# Autodesk Inventor assembly: Shooter Assembly
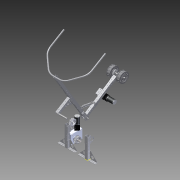
[picture p0: Inventor's stored thumbnail of the model, 180x180]
Saved by Autodesk Inventor 2014 (Build 180170000, 170)
## iProperties
Created: 2014-01-05
Part Number: Shooter Assembly
Document SubType Name: Assembly
Designer: Andrew Toennies
Mass: 7781.82 g
Surface Area: 22307.5 cm^2
Volume: 3128.72 cm^3
Density: 2.48722 g/cm^3
Author: Andrew Toennies
## Documents named in this file (34)
- C:\Users\Andrew Toennies\Documents\GitHub\2014buildCAD\Shooter\Shooter Assembly.iam
- C:\Users\Andrew Toennies\Documents\GitHub\2014buildCAD\Shooter\Vex Pro 1x1 rectangular tubing 12 in length.ipt
- C:\Users\Andrew Toennies\Documents\GitHub\2014buildCAD\Shooter\Vex Pro End Bearing Mount.ipt
- C:\Users\Andrew Toennies\Documents\GitHub\2014buildCAD\Shooter\Vex Pro 1x1 rectangular tubing 27 in length.ipt
- C:\Users\Andrew Toennies\Documents\GitHub\2014buildCAD\Shooter\Vex Pro 1x1 rectangular tubing 24 in length.ipt
- C:\Users\Andrew Toennies\Documents\GitHub\2014buildCAD\Shooter\Vex Pro Corner Gusset.ipt
- C:\Users\Andrew Toennies\Documents\GitHub\2014buildCAD\Shooter\Vex Pro 1x1 rectangular tubing 13 in length.ipt
- C:\Users\Andrew Toennies\Documents\GitHub\2014buildCAD\Shooter\Bearing ID 0.500 Hex OD 1.125.ipt
- C:\Users\Andrew Toennies\Documents\GitHub\2014buildCAD\Shooter\Axle 0.500 Hex 5 in length.ipt
- C:\Users\Andrew Toennies\Documents\GitHub\2014buildCAD\Shooter\Spacer.ipt
- C:\Users\Andrew Toennies\Documents\GitHub\2014buildCAD\Shooter\Bearing ID 0.375 OD 1.125.ipt
- C:\Users\Andrew Toennies\Documents\GitHub\2014buildCAD\Shooter\Axle 0.375 3 in length.ipt
- C:\Users\Andrew Toennies\Documents\GitHub\2014buildCAD\Shooter\Vex Pro 30 tooth 9mm timing belt pulley.ipt
- C:\Users\Andrew Toennies\Documents\GitHub\2014buildCAD\Shooter\Vex Pro VersaHub 0.500 Hex.ipt
- C:\Users\Andrew Toennies\Documents\GitHub\2014buildCAD\Shooter\Axle 0.500 Hex 3 in length.ipt
- C:\Users\Andrew Toennies\Documents\GitHub\2014buildCAD\Shooter\Worm-Drive-Gearbox-16to1.iam
- C:\Users\Andrew Toennies\Documents\GitHub\2014buildCAD\Shooter\Vex Pro 32 tooth 15 mm timing belt pulley.ipt
- C:\Users\Andrew Toennies\Documents\GitHub\2014buildCAD\Shooter\Vex Pro Traction 1 in wide 4 in dia wheel.iam
- C:\Users\Andrew Toennies\Documents\GitHub\2014buildCAD\Shooter\Aluminum Tube Bent 0.500 OD 0.436 ID.ipt
- C:\Users\Andrew Toennies\Documents\GitHub\2014buildCAD\Shooter\Bag Motor with VersaPlanetary 10 to 1 Reduction.iam
- C:\Users\Andrew Toennies\Documents\GitHub\2014buildCAD\Shooter\Vex Pro 18 tooth timing belt pulley.ipt
- C:\Users\Andrew Toennies\Documents\GitHub\2014buildCAD\Shooter\Vex Pro VersaPlanetary Face Mount.ipt
- C:\Users\Andrew Toennies\Documents\GitHub\2014buildCAD\Shooter\Foot Bracket Mount (McMaster Part #6498K710).ipt
- C:\Users\Andrew Toennies\Documents\GitHub\2014buildCAD\Shooter\Rod End (McMaster Part #6498K592).ipt
- C:\Users\Andrew Toennies\Documents\GitHub\2014buildCAD\Shooter\Spacer2.ipt
- C:\Users\Andrew Toennies\Documents\GitHub\2014buildCAD\Shooter\Bracket.ipt
- C:\Users\Andrew Toennies\Documents\GitHub\2014buildCAD\Shooter\Vex Pro 1x1 rectangular tubing 2 in length.ipt
- C:\Users\Andrew Toennies\Documents\GitHub\2014buildCAD\Shooter\Waterjetted Face Mount Bearing support VersaPlanetary.ipt
- C:\Users\Andrew Toennies\Documents\GitHub\2014buildCAD\Shooter\Axle 0.190 in 3 in length.ipt
- C:\Users\Andrew Toennies\Documents\GitHub\2014buildCAD\Shooter\6498K602 Pneumatic Cylinder Assembly.iam
- C:\Users\Andrew Toennies\Documents\GitHub\2014buildCAD\Shooter\mcmaster carr 32 tooth pulley.ipt
- C:\Users\Andrew Toennies\Documents\GitHub\2014buildCAD\Shooter\Vex Pro 1x1 rectangular tubing 4 in length.ipt
- C:\Users\Andrew Toennies\Documents\GitHub\2014buildCAD\Shooter\Vex Pro VersaFrame 90 Degree.ipt
- C:\Users\Andrew Toennies\Documents\GitHub\2014buildCAD\Shooter\Ball.ipt
## Components (59 placed, 33 different names)
1. Vex Pro Corner Gusset:1 — Insert:9, Insert:10, Mate:217, Flush:60, Flush:61
2. Vex Pro Corner Gusset:2 — Insert:11, Insert:12, Flush:50, Mate:216, Flush:78
3. Vex Pro End Bearing Mount:3 — Insert:35, Insert:47, Insert:48
4. Vex Pro End Bearing Mount:4 — Insert:36, Insert:49, Insert:50
5. Vex Pro End Bearing Mount:5 — Insert:21, Insert:22, Insert:25
6. Vex Pro End Bearing Mount:6 — Insert:23, Insert:24, Insert:26
7. Bearing ID 0.500 Hex OD 1.125:1 — Insert:26, Flush:7, Mate:7, Mate:8
8. Bearing ID 0.500 Hex OD 1.125:2 — Insert:25, Flush:7, Mate:16
9. Axle 0.500 Hex 5 in length:1 — Mate:7, Mate:8, Flush:8, Mate:14, Mate:15, Mate:18, Mate:19, Mate:21, Mate:22, Flush:12, Flush:16
10. Spacer:1 — Insert:47, Insert:48, Mate:65, Flush:24
11. Spacer:2 — Insert:49, Insert:50, Flush:22, Flush:23, Mate:64
12. Bearing ID 0.375 OD 1.125:1 — Insert:35, Mate:9
13. Bearing ID 0.375 OD 1.125:2 — Insert:36, Mate:66
14. Axle 0.375 3 in length:1 — Mate:9, Flush:9, Mate:66, Mate:85
15. Vex Pro 30 tooth 9mm timing belt pulley:1 — Mate:14, Mate:15, Mate:16, Flush:18
16. Vex Pro VersaHub 0.500 Hex:1 — Mate:17, Mate:18, Mate:19, Flush:16, Insert:51, Mate:105
17. Vex Pro VersaHub 0.500 Hex:2 — Mate:17, Mate:105
18. Vex Pro VersaHub 0.500 Hex:3 — Mate:20, Mate:21, Mate:22, Flush:12, Mate:52, Insert:64
19. Vex Pro VersaHub 0.500 Hex:4 — Mate:20, Mate:52, Insert:52
20. Axle 0.500 Hex 3 in length:1 — Mate:47, Mate:48, Mate:210, Mate:211, Flush:58, Flush:59
21. Worm-Drive-Gearbox-16to1:1 [sub-assembly] — Mate:49, Mate:50, Mate:170, Mate:196
22. Vex Pro 32 tooth 15 mm timing belt pulley:1 — Mate:47, Mate:48, Flush:40, Rotation:1
23. Vex Pro Traction 1 in wide 4 in dia wheel:1 [sub-assembly] — Insert:51
24. Vex Pro Traction 1 in wide 4 in dia wheel:2 [sub-assembly] — Insert:52, Insert:64
25. Aluminum Tube Bent 0.500 OD 0.436 ID:1 — Mate:53, Tangent:1, Tangent:2, Mate:230, Flush:80
26. Bag Motor with VersaPlanetary 10 to 1 Reduction:1 [sub-assembly] — Mate:55, Mate:56, Flush:19, Insert:53, Insert:54, Angle:4
27. Vex Pro 18 tooth timing belt pulley:1 — Mate:55, Mate:56, Flush:18
28. Vex Pro VersaPlanetary Face Mount:1 — Insert:53, Insert:54, Flush:21, Mate:63, Mate:77, Mate:78, Mate:79
29. Foot Bracket Mount (McMaster Part #6498K710):1 — Mate:71, Mate:72, Mate:73, Mate:99, Mate:100
30. Rod End (McMaster Part #6498K592):1 — Mate:102, Mate:103, Mate:194
31. Spacer2:1 — Mate:71, Mate:72, Mate:73, Mate:84, Mate:229
32. Bracket:1 — Mate:93, Mate:96, Flush:25, Flush:28, Flush:29
33. Bracket:2 — Mate:86, Mate:97, Flush:26, Flush:27
34. Waterjetted Face Mount Bearing support VersaPlanetary:1 — Mate:80, Mate:81, Mate:82, Insert:63
35. Bearing ID 0.500 Hex OD 1.125:5 — Insert:63, Angle:4
36. Axle 0.190 in 3 in length:1 — Mate:96, Mate:97, Flush:25, Mate:103
37. 6498K602 Pneumatic Cylinder Assembly:1 [sub-assembly] — Mate:99, Mate:100, Mate:102, Mate:194
38. mcmaster carr 32 tooth pulley:1 — Mate:170, Flush:40, Rotation:1
39. Vex Pro Corner Gusset:6 — Mate:182, Mate:183, Flush:45, Mate:231
40. Vex Pro Corner Gusset:7 — Flush:49, Flush:50, Mate:216, Mate:220, Flush:68, Flush:78
41. Vex Pro Corner Gusset:8 — Flush:49, Mate:221, Flush:68, Flush:69, Flush:70
42. Bearing ID 0.500 Hex OD 1.125:4 — Flush:57, Mate:210, Flush:59
43. Bearing ID 0.500 Hex OD 1.125:3 — Flush:55
44. Bearing ID 0.500 Hex OD 1.125:6 — Flush:55, Flush:56, Flush:58
45. Bearing ID 0.500 Hex OD 1.125:7 — Flush:56, Flush:57, Mate:211
46. Vex Pro Corner Gusset:9 — Mate:217, Flush:60, Flush:61, Flush:64, Flush:65, Mate:218, Flush:66, Flush:67
47. Vex Pro Corner Gusset:10 — Flush:64, Flush:65, Mate:219
48. Vex Pro VersaFrame 90 Degree:1 — Mate:222, Flush:71, Mate:223, Mate:227
49. Vex Pro VersaFrame 90 Degree:2 — Mate:224, Flush:72, Flush:73
50. Vex Pro VersaFrame 90 Degree:3 — Mate:225, Flush:74, Flush:75
51. Vex Pro VersaFrame 90 Degree:4 — Mate:226, Flush:76, Flush:77
52. Ball:1 — Tangent:1, Tangent:2
53. Vex Pro 1x1 rectangular tubing 2 in length:1 — Mate:77, Mate:78, Mate:79, Mate:80, Mate:81, Mate:82
54. Vex Pro 1x1 rectangular tubing 4 in length:2 — Mate:220, Mate:221, Flush:69, Flush:70, Mate:222, Flush:71, Mate:223, Mate:224, Flush:72, Flush:73
55. Vex Pro 1x1 rectangular tubing 4 in length:1 — Mate:218, Flush:66, Flush:67, Mate:219, Mate:225, Flush:74, Flush:75, Mate:226, Flush:76, Flush:77
56. Vex Pro 1x1 rectangular tubing 12 in length:1 — Insert:9, Insert:10, Insert:11, Insert:12, Mate:49, Mate:50, Mate:196
57. Vex Pro 1x1 rectangular tubing 27 in length:1 — Flush:2, Mate:2, Mate:182, Flush:45, Mate:227
58. Vex Pro 1x1 rectangular tubing 24 in length:1 — Flush:2, Mate:2, Flush:3, Flush:9, Mate:53, Flush:22, Flush:23, Mate:64, Mate:65, Flush:24, Mate:84, Mate:183, Mate:229, Mate:230, Mate:231, Flush:79
59. Vex Pro 1x1 rectangular tubing 13 in length:1 — Flush:3, Insert:21, Insert:22, Insert:23, Insert:24, Flush:8, Flush:19, Flush:21, Mate:63, Mate:85, Mate:86, Mate:93, Flush:26, Flush:27, Flush:28, Flush:29
## Relationships (139: Mate 67, Flush 46, Insert 22, Tangent 2, Angle 1, RelateRotation 1)
- Flush:2: Vex Pro 1x1 rectangular tubing 27 in length:1 ↔ Vex Pro 1x1 rectangular tubing 24 in length:1
- Mate:2: Vex Pro 1x1 rectangular tubing 27 in length:1 ↔ Vex Pro 1x1 rectangular tubing 24 in length:1
- Insert:9: Vex Pro Corner Gusset:1 ↔ Vex Pro 1x1 rectangular tubing 12 in length:1
- Insert:10: Vex Pro Corner Gusset:1 ↔ Vex Pro 1x1 rectangular tubing 12 in length:1
- Insert:11: Vex Pro Corner Gusset:2 ↔ Vex Pro 1x1 rectangular tubing 12 in length:1
- Insert:12: Vex Pro Corner Gusset:2 ↔ Vex Pro 1x1 rectangular tubing 12 in length:1
- Flush:3: Vex Pro 1x1 rectangular tubing 24 in length:1 ↔ Vex Pro 1x1 rectangular tubing 13 in length:1
- Insert:21: Vex Pro End Bearing Mount:5 ↔ Vex Pro 1x1 rectangular tubing 13 in length:1
- Insert:22: Vex Pro End Bearing Mount:5 ↔ Vex Pro 1x1 rectangular tubing 13 in length:1
- Insert:23: Vex Pro End Bearing Mount:6 ↔ Vex Pro 1x1 rectangular tubing 13 in length:1
- Insert:24: Vex Pro End Bearing Mount:6 ↔ Vex Pro 1x1 rectangular tubing 13 in length:1
- Insert:25: Vex Pro End Bearing Mount:5 ↔ Bearing ID 0.500 Hex OD 1.125:2
- Insert:26: Vex Pro End Bearing Mount:6 ↔ Bearing ID 0.500 Hex OD 1.125:1
- Flush:7: Bearing ID 0.500 Hex OD 1.125:1 ↔ Bearing ID 0.500 Hex OD 1.125:2
- Mate:7: Bearing ID 0.500 Hex OD 1.125:1 ↔ Axle 0.500 Hex 5 in length:1
- Mate:8: Bearing ID 0.500 Hex OD 1.125:1 ↔ Axle 0.500 Hex 5 in length:1
- Flush:8 (-63.5 mm): Axle 0.500 Hex 5 in length:1 ↔ Vex Pro 1x1 rectangular tubing 13 in length:1
- Insert:35: Vex Pro End Bearing Mount:3 ↔ Bearing ID 0.375 OD 1.125:1
- Insert:36: Vex Pro End Bearing Mount:4 ↔ Bearing ID 0.375 OD 1.125:2
- Mate:9: Bearing ID 0.375 OD 1.125:1 ↔ Axle 0.375 3 in length:1
- Flush:9 (-25.4 mm): Axle 0.375 3 in length:1 ↔ Vex Pro 1x1 rectangular tubing 24 in length:1
- Mate:14: Axle 0.500 Hex 5 in length:1 ↔ Vex Pro 30 tooth 9mm timing belt pulley:1
- Mate:15: Axle 0.500 Hex 5 in length:1 ↔ Vex Pro 30 tooth 9mm timing belt pulley:1
- Mate:16: Bearing ID 0.500 Hex OD 1.125:2 ↔ Vex Pro 30 tooth 9mm timing belt pulley:1
- Mate:17: Vex Pro VersaHub 0.500 Hex:1 ↔ Vex Pro VersaHub 0.500 Hex:2
- Mate:18: Axle 0.500 Hex 5 in length:1 ↔ Vex Pro VersaHub 0.500 Hex:1
- Mate:19: Axle 0.500 Hex 5 in length:1 ↔ Vex Pro VersaHub 0.500 Hex:1
- Mate:20: Vex Pro VersaHub 0.500 Hex:3 ↔ Vex Pro VersaHub 0.500 Hex:4
- Mate:21: Axle 0.500 Hex 5 in length:1 ↔ Vex Pro VersaHub 0.500 Hex:3
- Mate:22: Axle 0.500 Hex 5 in length:1 ↔ Vex Pro VersaHub 0.500 Hex:3
- Flush:12 (9.525 mm): Axle 0.500 Hex 5 in length:1 ↔ Vex Pro VersaHub 0.500 Hex:3
- Flush:16 (12.7 mm): Axle 0.500 Hex 5 in length:1 ↔ Vex Pro VersaHub 0.500 Hex:1
- Mate:47: Axle 0.500 Hex 3 in length:1 ↔ Vex Pro 32 tooth 15 mm timing belt pulley:1
- Mate:48: Axle 0.500 Hex 3 in length:1 ↔ Vex Pro 32 tooth 15 mm timing belt pulley:1
- Mate:49: Worm-Drive-Gearbox-16to1:1 ↔ Vex Pro 1x1 rectangular tubing 12 in length:1
- Mate:50: Worm-Drive-Gearbox-16to1:1 ↔ Vex Pro 1x1 rectangular tubing 12 in length:1
- Insert:47: Vex Pro End Bearing Mount:3 ↔ Spacer:1
- Insert:48: Vex Pro End Bearing Mount:3 ↔ Spacer:1
- Insert:49: Vex Pro End Bearing Mount:4 ↔ Spacer:2
- Insert:50: Vex Pro End Bearing Mount:4 ↔ Spacer:2
- Mate:52: Vex Pro VersaHub 0.500 Hex:3 ↔ Vex Pro VersaHub 0.500 Hex:4
- Insert:51: Vex Pro VersaHub 0.500 Hex:1 ↔ Vex Pro Traction 1 in wide 4 in dia wheel:1
- Insert:52: Vex Pro VersaHub 0.500 Hex:4 ↔ Vex Pro Traction 1 in wide 4 in dia wheel:2
- Mate:53: Aluminum Tube Bent 0.500 OD 0.436 ID:1 ↔ Vex Pro 1x1 rectangular tubing 24 in length:1
- Mate:55: Bag Motor with VersaPlanetary 10 to 1 Reduction:1 ↔ Vex Pro 18 tooth timing belt pulley:1
- Mate:56: Bag Motor with VersaPlanetary 10 to 1 Reduction:1 ↔ Vex Pro 18 tooth timing belt pulley:1
- Flush:18: Vex Pro 30 tooth 9mm timing belt pulley:1 ↔ Vex Pro 18 tooth timing belt pulley:1
- Flush:19: Bag Motor with VersaPlanetary 10 to 1 Reduction:1 ↔ Vex Pro 1x1 rectangular tubing 13 in length:1
- Insert:53: Bag Motor with VersaPlanetary 10 to 1 Reduction:1 ↔ Vex Pro VersaPlanetary Face Mount:1
- Insert:54: Bag Motor with VersaPlanetary 10 to 1 Reduction:1 ↔ Vex Pro VersaPlanetary Face Mount:1
- Flush:21: Vex Pro VersaPlanetary Face Mount:1 ↔ Vex Pro 1x1 rectangular tubing 13 in length:1
- Mate:63: Vex Pro VersaPlanetary Face Mount:1 ↔ Vex Pro 1x1 rectangular tubing 13 in length:1
- Flush:22: Spacer:2 ↔ Vex Pro 1x1 rectangular tubing 24 in length:1
- Flush:23: Spacer:2 ↔ Vex Pro 1x1 rectangular tubing 24 in length:1
- Mate:64: Spacer:2 ↔ Vex Pro 1x1 rectangular tubing 24 in length:1
- Mate:65: Spacer:1 ↔ Vex Pro 1x1 rectangular tubing 24 in length:1
- Flush:24: Spacer:1 ↔ Vex Pro 1x1 rectangular tubing 24 in length:1
- Mate:66: Bearing ID 0.375 OD 1.125:2 ↔ Axle 0.375 3 in length:1
- Mate:71: Foot Bracket Mount (McMaster Part #6498K710):1 ↔ Spacer2:1
- Mate:72: Foot Bracket Mount (McMaster Part #6498K710):1 ↔ Spacer2:1
- Mate:73: Foot Bracket Mount (McMaster Part #6498K710):1 ↔ Spacer2:1
- Mate:77: Vex Pro VersaPlanetary Face Mount:1 ↔ Vex Pro 1x1 rectangular tubing 2 in length:1
- Mate:78: Vex Pro VersaPlanetary Face Mount:1 ↔ Vex Pro 1x1 rectangular tubing 2 in length:1
- Mate:79: Vex Pro VersaPlanetary Face Mount:1 ↔ Vex Pro 1x1 rectangular tubing 2 in length:1
- Mate:80: Waterjetted Face Mount Bearing support VersaPlanetary:1 ↔ Vex Pro 1x1 rectangular tubing 2 in length:1
- Mate:81: Waterjetted Face Mount Bearing support VersaPlanetary:1 ↔ Vex Pro 1x1 rectangular tubing 2 in length:1
- Mate:82: Waterjetted Face Mount Bearing support VersaPlanetary:1 ↔ Vex Pro 1x1 rectangular tubing 2 in length:1
- Insert:63: Waterjetted Face Mount Bearing support VersaPlanetary:1 ↔ Bearing ID 0.500 Hex OD 1.125:5
- Angle:4 (0 deg): Bag Motor with VersaPlanetary 10 to 1 Reduction:1 ↔ Bearing ID 0.500 Hex OD 1.125:5
- Mate:84: Spacer2:1 ↔ Vex Pro 1x1 rectangular tubing 24 in length:1
- Insert:64: Vex Pro VersaHub 0.500 Hex:3 ↔ Vex Pro Traction 1 in wide 4 in dia wheel:2
- Mate:85: Axle 0.375 3 in length:1 ↔ Vex Pro 1x1 rectangular tubing 13 in length:1
- Mate:86: Bracket:2 ↔ Vex Pro 1x1 rectangular tubing 13 in length:1
- Mate:93: Bracket:1 ↔ Vex Pro 1x1 rectangular tubing 13 in length:1
- Mate:96: Bracket:1 ↔ Axle 0.190 in 3 in length:1
- Mate:97: Bracket:2 ↔ Axle 0.190 in 3 in length:1
- Flush:25 (-11.1125 mm): Bracket:1 ↔ Axle 0.190 in 3 in length:1
- Flush:26: Bracket:2 ↔ Vex Pro 1x1 rectangular tubing 13 in length:1
- Flush:27 (109.22 mm): Bracket:2 ↔ Vex Pro 1x1 rectangular tubing 13 in length:1
- Flush:28 (109.22 mm): Bracket:1 ↔ Vex Pro 1x1 rectangular tubing 13 in length:1
- Flush:29: Bracket:1 ↔ Vex Pro 1x1 rectangular tubing 13 in length:1
- Mate:99: Foot Bracket Mount (McMaster Part #6498K710):1 ↔ 6498K602 Pneumatic Cylinder Assembly:1
- Mate:100: Foot Bracket Mount (McMaster Part #6498K710):1 ↔ 6498K602 Pneumatic Cylinder Assembly:1
- Mate:102: Rod End (McMaster Part #6498K592):1 ↔ 6498K602 Pneumatic Cylinder Assembly:1
- Mate:103: Rod End (McMaster Part #6498K592):1 ↔ Axle 0.190 in 3 in length:1
- Mate:105: Vex Pro VersaHub 0.500 Hex:1 ↔ Vex Pro VersaHub 0.500 Hex:2
- Mate:170: Worm-Drive-Gearbox-16to1:1 ↔ mcmaster carr 32 tooth pulley:1
- Flush:40: Vex Pro 32 tooth 15 mm timing belt pulley:1 ↔ mcmaster carr 32 tooth pulley:1
- Rotation:1 [RelateRotation] (1 ul): Vex Pro 32 tooth 15 mm timing belt pulley:1 ↔ mcmaster carr 32 tooth pulley:1
- Mate:182: Vex Pro Corner Gusset:6 ↔ Vex Pro 1x1 rectangular tubing 27 in length:1
- Mate:183: Vex Pro Corner Gusset:6 ↔ Vex Pro 1x1 rectangular tubing 24 in length:1
- Flush:45: Vex Pro Corner Gusset:6 ↔ Vex Pro 1x1 rectangular tubing 27 in length:1
- Mate:194 (-12.7 mm): Rod End (McMaster Part #6498K592):1 ↔ 6498K602 Pneumatic Cylinder Assembly:1
- Mate:196: Worm-Drive-Gearbox-16to1:1 ↔ Vex Pro 1x1 rectangular tubing 12 in length:1
- Flush:49: Vex Pro Corner Gusset:7 ↔ Vex Pro Corner Gusset:8
- Flush:50: Vex Pro Corner Gusset:2 ↔ Vex Pro Corner Gusset:7
- Flush:55: Bearing ID 0.500 Hex OD 1.125:3 ↔ Bearing ID 0.500 Hex OD 1.125:6
- Flush:56: Bearing ID 0.500 Hex OD 1.125:6 ↔ Bearing ID 0.500 Hex OD 1.125:7
- Flush:57: Bearing ID 0.500 Hex OD 1.125:4 ↔ Bearing ID 0.500 Hex OD 1.125:7
- Mate:210: Axle 0.500 Hex 3 in length:1 ↔ Bearing ID 0.500 Hex OD 1.125:4
- Mate:211: Axle 0.500 Hex 3 in length:1 ↔ Bearing ID 0.500 Hex OD 1.125:7
- Flush:58: Axle 0.500 Hex 3 in length:1 ↔ Bearing ID 0.500 Hex OD 1.125:6
- Flush:59: Axle 0.500 Hex 3 in length:1 ↔ Bearing ID 0.500 Hex OD 1.125:4
- Mate:216 (50.8 mm): Vex Pro Corner Gusset:2 ↔ Vex Pro Corner Gusset:7
- Mate:217: Vex Pro Corner Gusset:1 ↔ Vex Pro Corner Gusset:9
- Flush:60: Vex Pro Corner Gusset:1 ↔ Vex Pro Corner Gusset:9
- Flush:61: Vex Pro Corner Gusset:1 ↔ Vex Pro Corner Gusset:9
- Flush:64: Vex Pro Corner Gusset:9 ↔ Vex Pro Corner Gusset:10
- Flush:65: Vex Pro Corner Gusset:9 ↔ Vex Pro Corner Gusset:10
- Mate:218: Vex Pro Corner Gusset:9 ↔ Vex Pro 1x1 rectangular tubing 4 in length:1
- Flush:66: Vex Pro Corner Gusset:9 ↔ Vex Pro 1x1 rectangular tubing 4 in length:1
- Flush:67: Vex Pro Corner Gusset:9 ↔ Vex Pro 1x1 rectangular tubing 4 in length:1
- Mate:219: Vex Pro Corner Gusset:10 ↔ Vex Pro 1x1 rectangular tubing 4 in length:1
- Mate:220: Vex Pro Corner Gusset:7 ↔ Vex Pro 1x1 rectangular tubing 4 in length:2
- Mate:221: Vex Pro Corner Gusset:8 ↔ Vex Pro 1x1 rectangular tubing 4 in length:2
- Flush:68: Vex Pro Corner Gusset:7 ↔ Vex Pro Corner Gusset:8
- Flush:69: Vex Pro Corner Gusset:8 ↔ Vex Pro 1x1 rectangular tubing 4 in length:2
- Flush:70: Vex Pro Corner Gusset:8 ↔ Vex Pro 1x1 rectangular tubing 4 in length:2
- Mate:222: Vex Pro VersaFrame 90 Degree:1 ↔ Vex Pro 1x1 rectangular tubing 4 in length:2
- Flush:71: Vex Pro VersaFrame 90 Degree:1 ↔ Vex Pro 1x1 rectangular tubing 4 in length:2
- Mate:223: Vex Pro VersaFrame 90 Degree:1 ↔ Vex Pro 1x1 rectangular tubing 4 in length:2
- Mate:224: Vex Pro VersaFrame 90 Degree:2 ↔ Vex Pro 1x1 rectangular tubing 4 in length:2
- Flush:72: Vex Pro VersaFrame 90 Degree:2 ↔ Vex Pro 1x1 rectangular tubing 4 in length:2
- Flush:73: Vex Pro VersaFrame 90 Degree:2 ↔ Vex Pro 1x1 rectangular tubing 4 in length:2
- Mate:225: Vex Pro VersaFrame 90 Degree:3 ↔ Vex Pro 1x1 rectangular tubing 4 in length:1
- Flush:74: Vex Pro VersaFrame 90 Degree:3 ↔ Vex Pro 1x1 rectangular tubing 4 in length:1
- Flush:75: Vex Pro VersaFrame 90 Degree:3 ↔ Vex Pro 1x1 rectangular tubing 4 in length:1
- Mate:226: Vex Pro VersaFrame 90 Degree:4 ↔ Vex Pro 1x1 rectangular tubing 4 in length:1
- Flush:76: Vex Pro VersaFrame 90 Degree:4 ↔ Vex Pro 1x1 rectangular tubing 4 in length:1
- Flush:77: Vex Pro VersaFrame 90 Degree:4 ↔ Vex Pro 1x1 rectangular tubing 4 in length:1
- Mate:227: Vex Pro VersaFrame 90 Degree:1 ↔ Vex Pro 1x1 rectangular tubing 27 in length:1
- Flush:78: Vex Pro Corner Gusset:2 ↔ Vex Pro Corner Gusset:7
- Tangent:1: Aluminum Tube Bent 0.500 OD 0.436 ID:1 ↔ Ball:1
- Tangent:2: Aluminum Tube Bent 0.500 OD 0.436 ID:1 ↔ Ball:1
- Mate:229: Spacer2:1 ↔ Vex Pro 1x1 rectangular tubing 24 in length:1
- Mate:230 (-12.7 mm): Aluminum Tube Bent 0.500 OD 0.436 ID:1 ↔ Vex Pro 1x1 rectangular tubing 24 in length:1
- Mate:231: Vex Pro Corner Gusset:6 ↔ Vex Pro 1x1 rectangular tubing 24 in length:1
- Flush:79 (330.2 mm): Vex Pro 1x1 rectangular tubing 24 in length:1
- Flush:80: Aluminum Tube Bent 0.500 OD 0.436 ID:1
